# Autodesk Inventor assembly: Base Design 2
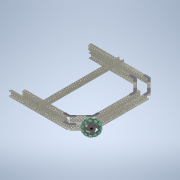
[picture p0: Inventor's stored thumbnail of the model, 180x180]
Saved by Autodesk Inventor 2020 (Build 240168000, 168)
## iProperties
Created: 2019-08-27
Part Number: Base Design 2
Document SubType Name: Assembly
Designer: spenc
Author: spenc
## Documents named in this file (9)
- C:\Users\Corey\Google Drive\2019_2020 Tower Takeover\CAD\Base Design 2.iam
- C:\Users\Corey\Google Drive\2019_2020 Tower Takeover\CAD\Parts\Structure\C-Channels\Aluminum\2-Wide\Aluminum C-Channel 1x2x1x25.ipt
- C:\Users\Corey\Google Drive\2019_2020 Tower Takeover\CAD\Parts\Structure\Gussets\45 Degree Gusset.ipt
- C:\Users\Corey\Google Drive\2019_2020 Tower Takeover\CAD\Parts\Structure\C-Channels\Aluminum\2-Wide\Aluminum C-Channel 1x2x1x35.ipt
- C:\Users\Corey\Google Drive\2019_2020 Tower Takeover\CAD\Parts\Structure\C-Channels\Aluminum\2-Wide\Aluminum C-Channel 1x2x1x19.ipt
- C:\Users\Corey\Google Drive\2019_2020 Tower Takeover\CAD\Parts\Structure\C-Channels\Aluminum\2-Wide\Aluminum C-Channel 1x2x1x6.ipt
- C:\Users\Corey\Google Drive\2019_2020 Tower Takeover\CAD\Parts\Structure\C-Channels\Aluminum\2-Wide\Aluminum C-Channel 1x2x1x22.ipt
- C:\Users\Corey\Google Drive\2019_2020 Tower Takeover\CAD\Parts\Motion\Wheels & Rollers\3.25'' Omni-Directional Wheel, Square Insert.iam
- C:\Users\Corey\Google Drive\2019_2020 Tower Takeover\CAD\Parts\Structure\C-Channels\Aluminum\2-Wide\Aluminum C-Channel 1x2x1x7.ipt
## Components (20 placed, 8 different names)
1. Aluminum C-Channel 1x2x1x25:4 — Mate:1, Flush:1, Mate:2, Flush:2, Flush:13, Flush:15, Insert:3
2. 45 Degree Gusset:1 — Mate:4, Flush:3, Insert:2, Mate:22, Flush:22, Insert:11
3. 45 Degree Gusset:3 — Mate:1, Flush:1, Mate:8, Mate:9, Insert:3, Insert:4
4. Aluminum C-Channel 1x2x1x35:1 — Mate:2, Flush:2, Mate:3, Mate:12, Mate:13, Flush:6, Flush:12, Flush:13, Flush:14, Flush:15, Flush:16, Flush:17, Flush:18, Flush:19
5. Aluminum C-Channel 1x2x1x19:1 — Mate:3, Mate:4, Flush:3, Flush:12, Flush:14, Insert:2
6. Aluminum C-Channel 1x2x1x6:3 — Mate:8, Mate:9, Mate:10, Flush:4, Insert:4
7. 45 Degree Gusset:4 — Mate:10, Flush:4, Mate:21, Flush:21
8. 45 Degree Gusset:5 — Mate:20, Flush:20, Mate:23, Flush:23, Insert:12, Insert:13
9. Aluminum C-Channel 1x2x1x19:3 — Mate:12, Mate:15, Flush:8, Flush:18, Flush:19, Insert:10
10. Aluminum C-Channel 1x2x1x25:5 — Mate:13, Flush:6, Mate:14, Flush:7, Flush:16, Flush:17, Insert:7
11. 45 Degree Gusset:6 — Mate:14, Flush:7, Mate:16, Flush:9, Insert:7, Insert:8
12. 45 Degree Gusset:7 — Mate:15, Flush:8, Insert:10, Mate:24, Flush:24, Insert:14
13. Aluminum C-Channel 1x2x1x6:4 — Mate:16, Flush:9, Mate:18, Insert:8
14. 45 Degree Gusset:8 — Mate:25, Flush:25, Insert:15
15. 45 Degree Gusset:9 — Mate:18
16. Aluminum C-Channel 1x2x1x19:4 — Mate:20, Flush:20, Insert:13
17. Aluminum C-Channel 1x2x1x22:1 — Mate:21, Flush:21
18. 3.25'' Omni-Directional Wheel, Square Insert:1 [sub-assembly]
19. Aluminum C-Channel 1x2x1x7:1 — Mate:22, Flush:22, Insert:11, Mate:23, Flush:23, Insert:12
20. Aluminum C-Channel 1x2x1x7:2 — Mate:24, Flush:24, Insert:14, Mate:25, Flush:25, Insert:15
## Relationships (52: Flush 22, Mate 19, Insert 11)
- Mate:1: Aluminum C-Channel 1x2x1x25:4 ↔ 45 Degree Gusset:3
- Flush:1: Aluminum C-Channel 1x2x1x25:4 ↔ 45 Degree Gusset:3
- Mate:2: Aluminum C-Channel 1x2x1x25:4 ↔ Aluminum C-Channel 1x2x1x35:1
- Flush:2: Aluminum C-Channel 1x2x1x25:4 ↔ Aluminum C-Channel 1x2x1x35:1
- Mate:3: Aluminum C-Channel 1x2x1x35:1 ↔ Aluminum C-Channel 1x2x1x19:1
- Mate:4: 45 Degree Gusset:1 ↔ Aluminum C-Channel 1x2x1x19:1
- Flush:3: 45 Degree Gusset:1 ↔ Aluminum C-Channel 1x2x1x19:1
- Mate:8: 45 Degree Gusset:3 ↔ Aluminum C-Channel 1x2x1x6:3
- Mate:9: 45 Degree Gusset:3 ↔ Aluminum C-Channel 1x2x1x6:3
- Mate:10: Aluminum C-Channel 1x2x1x6:3 ↔ 45 Degree Gusset:4
- Flush:4: Aluminum C-Channel 1x2x1x6:3 ↔ 45 Degree Gusset:4
- Mate:12: Aluminum C-Channel 1x2x1x35:1 ↔ Aluminum C-Channel 1x2x1x19:3
- Mate:13: Aluminum C-Channel 1x2x1x35:1 ↔ Aluminum C-Channel 1x2x1x25:5
- Flush:6: Aluminum C-Channel 1x2x1x35:1 ↔ Aluminum C-Channel 1x2x1x25:5
- Mate:14: Aluminum C-Channel 1x2x1x25:5 ↔ 45 Degree Gusset:6
- Flush:7: Aluminum C-Channel 1x2x1x25:5 ↔ 45 Degree Gusset:6
- Mate:15: Aluminum C-Channel 1x2x1x19:3 ↔ 45 Degree Gusset:7
- Flush:8: Aluminum C-Channel 1x2x1x19:3 ↔ 45 Degree Gusset:7
- Mate:16: 45 Degree Gusset:6 ↔ Aluminum C-Channel 1x2x1x6:4
- Flush:9: 45 Degree Gusset:6 ↔ Aluminum C-Channel 1x2x1x6:4
- Mate:18: Aluminum C-Channel 1x2x1x6:4 ↔ 45 Degree Gusset:9
- Flush:12: Aluminum C-Channel 1x2x1x35:1 ↔ Aluminum C-Channel 1x2x1x19:1
- Flush:13: Aluminum C-Channel 1x2x1x25:4 ↔ Aluminum C-Channel 1x2x1x35:1
- Flush:14: Aluminum C-Channel 1x2x1x35:1 ↔ Aluminum C-Channel 1x2x1x19:1
- Flush:15: Aluminum C-Channel 1x2x1x25:4 ↔ Aluminum C-Channel 1x2x1x35:1
- Insert:2: 45 Degree Gusset:1 ↔ Aluminum C-Channel 1x2x1x19:1
- Insert:3: Aluminum C-Channel 1x2x1x25:4 ↔ 45 Degree Gusset:3
- Insert:4: 45 Degree Gusset:3 ↔ Aluminum C-Channel 1x2x1x6:3
- Flush:16: Aluminum C-Channel 1x2x1x35:1 ↔ Aluminum C-Channel 1x2x1x25:5
- Flush:17: Aluminum C-Channel 1x2x1x35:1 ↔ Aluminum C-Channel 1x2x1x25:5
- Flush:18: Aluminum C-Channel 1x2x1x35:1 ↔ Aluminum C-Channel 1x2x1x19:3
- Flush:19: Aluminum C-Channel 1x2x1x35:1 ↔ Aluminum C-Channel 1x2x1x19:3
- Insert:7: Aluminum C-Channel 1x2x1x25:5 ↔ 45 Degree Gusset:6
- Insert:8: 45 Degree Gusset:6 ↔ Aluminum C-Channel 1x2x1x6:4
- Insert:10: Aluminum C-Channel 1x2x1x19:3 ↔ 45 Degree Gusset:7
- Mate:20: 45 Degree Gusset:5 ↔ Aluminum C-Channel 1x2x1x19:4
- Flush:20: 45 Degree Gusset:5 ↔ Aluminum C-Channel 1x2x1x19:4
- Mate:21: 45 Degree Gusset:4 ↔ Aluminum C-Channel 1x2x1x22:1
- Flush:21: 45 Degree Gusset:4 ↔ Aluminum C-Channel 1x2x1x22:1
- Mate:22: 45 Degree Gusset:1 ↔ Aluminum C-Channel 1x2x1x7:1
- Flush:22: 45 Degree Gusset:1 ↔ Aluminum C-Channel 1x2x1x7:1
- Insert:11: 45 Degree Gusset:1 ↔ Aluminum C-Channel 1x2x1x7:1
- Mate:23: 45 Degree Gusset:5 ↔ Aluminum C-Channel 1x2x1x7:1
- Flush:23: 45 Degree Gusset:5 ↔ Aluminum C-Channel 1x2x1x7:1
- Insert:12: 45 Degree Gusset:5 ↔ Aluminum C-Channel 1x2x1x7:1
- Insert:13: 45 Degree Gusset:5 ↔ Aluminum C-Channel 1x2x1x19:4
- Mate:24: 45 Degree Gusset:7 ↔ Aluminum C-Channel 1x2x1x7:2
- Flush:24: 45 Degree Gusset:7 ↔ Aluminum C-Channel 1x2x1x7:2
- Insert:14: 45 Degree Gusset:7 ↔ Aluminum C-Channel 1x2x1x7:2
- Mate:25: 45 Degree Gusset:8 ↔ Aluminum C-Channel 1x2x1x7:2
- Flush:25: 45 Degree Gusset:8 ↔ Aluminum C-Channel 1x2x1x7:2
- Insert:15: 45 Degree Gusset:8 ↔ Aluminum C-Channel 1x2x1x7:2
